# Autodesk Inventor assembly: Lepton 3 thermal camera
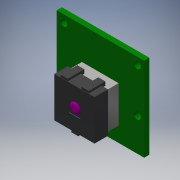
[picture p0: Inventor's stored thumbnail of the model, 180x180]
Saved by Autodesk Inventor 2018 (Build 220112000, 112)
## iProperties
Created: 2018-05-02
Part Number: Lepton 3 thermal camera
Document SubType Name: Assembly
Designer: Ajith Thomas
Author: Ajith Thomas
## Documents named in this file (3)
- C:\Users\Ajith Thomas\Dropbox\Gas_Sensing_Robot\FumeBot-Design\Sensors and Boards\Lepton 3 Thermal Camera\Lepton 3 thermal camera.iam
- C:\Users\Ajith Thomas\Dropbox\Gas_Sensing_Robot\FumeBot-Design\Sensors and Boards\Lepton 3 Thermal Camera\Breakout Board.ipt
- C:\Users\Ajith Thomas\Dropbox\Gas_Sensing_Robot\FumeBot-Design\Sensors and Boards\Lepton 3 Thermal Camera\Thermal module.ipt
## Components (2 placed, 2 different names)
1. Breakout Board:1 — Mate:1, Flush:1, Flush:2
2. Thermal module:1 — Mate:1, Flush:1, Flush:2
## Relationships (3: Flush 2, Mate 1)
- Mate:1: Breakout Board:1 ↔ Thermal module:1
- Flush:1 (8.091 mm): Breakout Board:1 ↔ Thermal module:1
- Flush:2 (6.782 mm): Breakout Board:1 ↔ Thermal module:1
